# Autodesk Inventor assembly: fb02
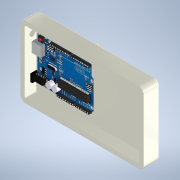
[picture p0: Inventor's stored thumbnail of the model, 180x180]
Saved by Autodesk Inventor 2021 (Build 250183000, 183)
## iProperties
Created: 2021-10-11
Part Number: fb02
Document SubType Name: Assembly
Designer: gonza
Author: gonza
## Documents named in this file (5)
- C:\Users\USUARIO\Dropbox\Mi PC (LAPTOP-MNA512CM)\Desktop\fb02.iam
- C:\Users\USUARIO\Dropbox\Mi PC (LAPTOP-MNA512CM)\Desktop\Biodiseño\ScreenCase.ipt
- C:\Users\USUARIO\Dropbox\Mi PC (LAPTOP-MNA512CM)\Desktop\Biodiseño\ardino.ipt
- C:\Users\gonza\OneDrive\Documentos\Inventor\Content Center Files\R2021\en-US\AS 1110\AS 1110 - M3 x 6.ipt
- C:\Users\gonza\OneDrive\Documentos\Inventor\Content Center Files\R2021\en-US\AS 1110\AS 1110 - M4 x 8.ipt
## Components (6 placed, 4 different names)
1. ScreenCase:1 — Mate:4, Mate:5, Mate:6, Mate:7, Mate:8, Mate:22, Mate:23
2. ardino:1 — Mate:6, Mate:7, Mate:8, Insert:1, Insert:2, Insert:3, Insert:4
3. AS 1110 - Metric M3 x 6:1 — Insert:1
4. AS 1110 - Metric M4 x 8:1 — Insert:2
5. AS 1110 - Metric M3 x 6:2 — Insert:3
6. AS 1110 - Metric M3 x 6:3 — Insert:4
## Relationships (11: Mate 7, Insert 4)
- Mate:4: ScreenCase:1
- Mate:5: ScreenCase:1
- Mate:6: ScreenCase:1 ↔ ardino:1
- Mate:7 (2.89 mm): ScreenCase:1 ↔ ardino:1
- Mate:8 (13 mm): ScreenCase:1 ↔ ardino:1
- Insert:1: ardino:1 ↔ AS 1110 - Metric M3 x 6:1
- Insert:2: ardino:1 ↔ AS 1110 - Metric M4 x 8:1
- Insert:3: ardino:1 ↔ AS 1110 - Metric M3 x 6:2
- Insert:4: ardino:1 ↔ AS 1110 - Metric M3 x 6:3
- Mate:22: ScreenCase:1
- Mate:23: ScreenCase:1
